# Autodesk Inventor assembly: SVWB
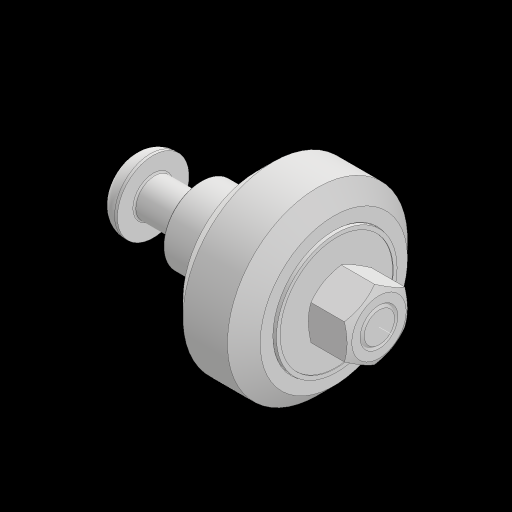
[picture p0: Inventor's stored thumbnail of the model, 512x512]
Saved by Autodesk Inventor 2023 (Build 270158000, 158)
## iProperties
Created: 2022-08-02
Part Number: SVWB
Document SubType Name: Assembly
Designer: tandu
Author: tandu
Revision Number: ANY
## Documents named in this file (5)
- C:\Users\tandu\Documents\GrabCAD\Custom Conveyor Belt 3D Printer\References\Roller based conveyor belt 3d printer\RollerVersionSVWB.iam
- C:\Users\tandu\Documents\GrabCAD\Custom Conveyor Belt 3D Printer\References\Roller based conveyor belt 3d printer\RollerVersionSVWB.iam.iam
- RollerVersionSVWB.iam
- SVWB.iam
- RollerVersionSolid V Wheel.ipt
## Components (1 placed, 1 different names)
1. SVWB.iam_78 [sub-assembly] — Mate:1, Flush:1
## Relationships (2: Mate 1, Flush 1)
- Mate:1: SVWB.iam_78
- Flush:1: SVWB.iam_78
